# Autodesk Inventor assembly: Assembly2
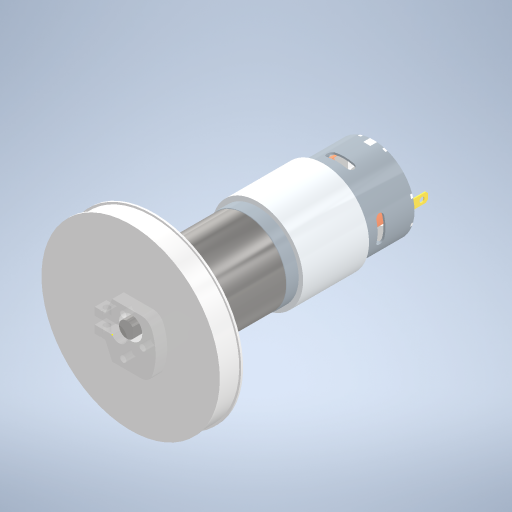
[picture p0: Inventor's stored thumbnail of the model, 512x512]
Saved by Autodesk Inventor 2023 (Build 270158000, 158)
## iProperties
Created: 2022-04-25
Part Number: Assembly2
Document SubType Name: Assembly
Designer: yuta
Author: yuta
## Documents named in this file (3)
- C:\Users\yuta\Documents\NHK\Assembly2.iam
- C:\Users\yuta\Documents\NHK\RS775+gennsoku.iam
- C:\Users\yuta\Documents\NHK\射出_本体.iam
## Components (2 placed, 2 different names)
1. RS775+gennsoku:1 [sub-assembly] — メイト:1, メイト:2
2. 射出_本体:1 [sub-assembly] — メイト:1, メイト:2
## Relationships (2: Mate 2)
- メイト:1 [Mate]: RS775+gennsoku:1 ↔ 射出_本体:1
- メイト:2 [Mate]: RS775+gennsoku:1 ↔ 射出_本体:1
